# Autodesk Inventor assembly: strecha sestava
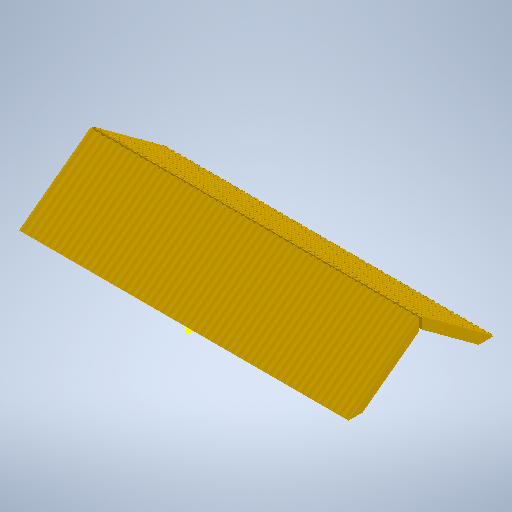
[picture p0: Inventor's stored thumbnail of the model, 512x512]
Saved by Autodesk Inventor 2025.1 (Build 291241000, 241)
## iProperties
Created: 2024-11-01
Part Number: strecha sestava
Document SubType Name: Assembly
Designer: nelan
Author: nelan
## Documents named in this file (3)
- C:\Users\nelan\Documents\Nelca\Škola\_projekt\navrh\strecha sestava.iam
- C:\Users\nelan\Documents\Nelca\Škola\_projekt\navrh\strecha.ipt
- C:\Users\nelan\Documents\Nelca\Škola\_projekt\navrh\strecha druha.ipt
## Components (2 placed, 2 different names)
1. strecha:1 — Proti sobě:1, Proti sobě:2
2. strecha druha:1 — Proti sobě:1, Proti sobě:2
## Relationships (2: Mate 2)
- Proti sobě:1 [Mate]: strecha:1 ↔ strecha druha:1
- Proti sobě:2 [Mate]: strecha:1 ↔ strecha druha:1
